# Autodesk Inventor assembly: Fisher Price Motor 1764
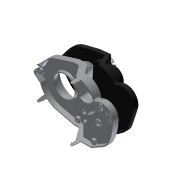
[picture p0: Inventor's stored thumbnail of the model, 180x180]
Saved by Autodesk Inventor 2011 (Build 150239000, 239)
## iProperties
Shininess: 64.0
Angle Display Precision: 2
Document Length Units: 11272
Document Angle Units: 11279
Document Time Units: 11290
Document Mass Units: 11286
Document Length Units Precision: 3
Document Angle Units Precision: 2
Category: Motors
Created: 2001-12-27
Document SubType Name: Assembly
Project: FIRST
Vendor: FisherPrice
Part Number: Fisher Price Motor 1764
Description: FisherPrice Motor and Gearbox
Density: 0.0
Volumn: 0.0
Area: 0.0
PropertySet Name: Model Information
Control State: 0
Master: False
Checked Out: False
Title: FisherPrice Motor and Gearbox
Author: Autodesk, Inc.
## Documents named in this file (4)
- R:\2010-2011\CMO\Web Site\CADalog\Motors\Fisher Price Motor Team 1764.iam
- R:\2009-2010\CAD\Motors\Fisher Price Window Motor Team 1764\Fisher Price Front Housing 1764.ipt
- R:\2009-2010\CAD\Motors\Fisher Price Window Motor Team 1764\Fisher Price Back Housing .ipt
- R:\2009-2010\CAD\Motors\Fisher Price Window Motor Team 1764\Motor Spindle.ipt
## Components (3 placed, 3 different names)
1. Fisher Price Front Housing 1764:1 — Flush:1, Flush:2, Mate:2, Mate:3
2. Fisher Price Back Housing :1 — Flush:1, Mate:1, Mate:2, Mate:3
3. Motor Spindle:1 — Flush:2, Mate:1
## Relationships (5: Mate 3, Flush 2)
- Flush:1: Fisher Price Front Housing 1764:1 ↔ Fisher Price Back Housing :1
- Flush:2: Fisher Price Front Housing 1764:1 ↔ Motor Spindle:1
- Mate:1: Fisher Price Back Housing :1 ↔ Motor Spindle:1
- Mate:2: Fisher Price Front Housing 1764:1 ↔ Fisher Price Back Housing :1
- Mate:3: Fisher Price Front Housing 1764:1 ↔ Fisher Price Back Housing :1
